# Autodesk Inventor assembly: front_panel
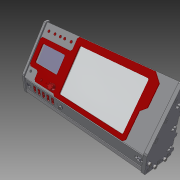
[picture p0: Inventor's stored thumbnail of the model, 180x180]
Saved by Autodesk Inventor 2014 (Build 180170000, 170)
## iProperties
Created: 2014-04-02
Part Number: front_panel
Document SubType Name: Assembly
Designer: buben
Author: buben
## Documents named in this file (20)
- C:\Users\buben\Documents\GitHub\bacon\inventor files\assemblies\front_panel.iam
- C:\Users\buben\Documents\GitHub\bacon\inventor files\printer parts\front_panel_brace_right.ipt
- C:\Users\buben\Documents\GitHub\bacon\inventor files\printer parts\front_panel_lcd.ipt
- C:\Users\buben\Documents\GitHub\bacon\inventor files\printer parts\front_panel_bottom.ipt
- C:\Users\buben\Documents\GitHub\bacon\inventor files\printer parts\front_panel_middle.ipt
- C:\Users\buben\Documents\GitHub\bacon\inventor files\printer parts\front_panel_brace_left.ipt
- C:\Users\buben\Documents\GitHub\bacon\inventor files\utils\washer_m4.ipt
- C:\Users\buben\Documents\Inventor\Content Center Files\R2014\en-US\ISO 4762(2)\ISO 4762 - M4 x 20ISO.ipt
- C:\Users\buben\Documents\Inventor\Content Center Files\R2014\en-US\ISO 7040\ISO 7040 - M4.ipt
- C:\Users\buben\Documents\GitHub\bacon\inventor files\printer parts\front_panel_brace_middle.ipt
- C:\Users\buben\Documents\GitHub\bacon\inventor files\utils\main_lcd_controller\lcd_controller.iam
- C:\Users\buben\Documents\GitHub\bacon\inventor files\utils\main_lcd_push_button.ipt
- C:\Users\buben\Documents\GitHub\bacon\inventor files\3rd party components\USB socket\Imported Components\USB-Socket\USB-Socket.ipt
- C:\Users\buben\Documents\GitHub\bacon\inventor files\utils\ramps_smart_controller\controler.iam
- C:\Users\buben\Documents\GitHub\bacon\inventor files\utils\controller_lcd_cover_glass.ipt
- C:\Users\buben\Documents\GitHub\bacon\inventor files\utils\main_lcd_panel.ipt
- C:\Users\buben\Documents\GitHub\bacon\inventor files\utils\main_lcd_cover_glass.ipt
- C:\Users\buben\Documents\GitHub\bacon\inventor files\utils\front_panel_frame.ipt
- C:\Users\buben\Documents\GitHub\bacon\inventor files\utils\controller_push_button.ipt
- C:\Users\buben\Documents\GitHub\bacon\inventor files\utils\rotary_encoder_cnob.ipt
## Components (56 placed, 19 different names)
1. front_panel_brace_right:1 — Flush:1, Mate:1, Mate:2, Mate:3, Mate:4, Mate:5, Mate:6, Mate:7, Mate:8, Mate:9, Flush:2, Flush:3, Mate:14, Mate:15, Mate:16, Mate:17, Mate:18, Mate:19
2. front_panel_lcd:1 — Mate:3, Mate:4, Mate:5, Mate:10, Mate:11, Mate:12, Mate:44, Angle:1, Mate:45, Mate:46, Mate:47, Mate:48, Mate:49, Mate:50, Flush:4, Mate:59, Mate:60, Flush:5, Mate:61, Mate:62, Mate:63, Flush:6, Mate:64, Flush:7, Mate:65, Mate:66, Mate:79, Mate:80
3. front_panel_bottom:1 — Mate:6, Mate:7, Mate:8, Mate:13, Mate:21, Mate:22, Mate:42, Mate:43, Mate:69, Mate:70
4. front_panel_middle:1 — Mate:9, Flush:2, Mate:10, Mate:20, Mate:41, Mate:56, Mate:57, Mate:58, Mate:67, Mate:68
5. front_panel_brace_left:1 — Mate:11, Mate:12, Mate:13
6. CSN 02 1702 B B 4,3:1 — Mate:15, Mate:18, Insert:2
7. CSN 02 1702 B B 4,3:2 — Mate:14, Mate:19, Insert:3
8. CSN 02 1702 B B 4,3:3 — Mate:16, Mate:17, Insert:1
9. CSN 02 1702 B B 4,3:4 — Mate:21, Mate:24, Mate:28
10. CSN 02 1702 B B 4,3:5 — Mate:22, Mate:25, Mate:30
11. CSN 02 1702 B B 4,3:6 — Mate:20, Mate:23, Mate:26
12. ISO 4762 M4 x 20:1 — Insert:1, Mate:23, Mate:27
13. ISO 4762 M4 x 20:2 — Insert:2, Mate:24, Mate:29
14. ISO 4762 M4 x 20:3 — Insert:3, Mate:25, Mate:31
15. DIN EN ISO 7040 M4:1 — Mate:30, Mate:31
16. DIN EN ISO 7040 M4:2 — Mate:28, Mate:29
17. DIN EN ISO 7040 M4:3 — Mate:26, Mate:27
18. CSN 02 1702 B B 4,3:7 — Insert:5
19. CSN 02 1702 B B 4,3:8 — Insert:6
20. CSN 02 1702 B B 4,3:9 — Insert:4
21. CSN 02 1702 B B 4,3:10 — Mate:33, Mate:38
22. CSN 02 1702 B B 4,3:11 — Mate:34, Mate:36
23. CSN 02 1702 B B 4,3:12 — Mate:32, Mate:40
24. ISO 4762 M4 x 20:4 — Mate:32, Insert:4, Mate:39
25. ISO 4762 M4 x 20:5 — Mate:33, Insert:5, Mate:37
26. ISO 4762 M4 x 20:6 — Mate:34, Insert:6, Mate:35
27. DIN EN ISO 7040 M4:4 — Mate:35, Mate:36
28. DIN EN ISO 7040 M4:5 — Mate:37, Mate:38
29. DIN EN ISO 7040 M4:6 — Mate:39, Mate:40
30. front_panel_brace_middle:1 — Mate:41, Mate:42, Mate:43, Mate:71, Mate:73
31. lcd_controller:1 [sub-assembly] — Mate:44, Angle:1, Mate:45, Mate:51, Mate:52, Mate:53, Mate:54, Mate:55
32. main_lcd_push_button:1 — Mate:46, Mate:55
33. main_lcd_push_button:2 — Mate:47, Mate:54
34. main_lcd_push_button:3 — Mate:48, Mate:53
35. main_lcd_push_button:4 — Mate:49, Mate:52
36. main_lcd_push_button:5 — Mate:50, Mate:51
37. controler:1 [sub-assembly] — Flush:4, Mate:59, Mate:60, Mate:81, Mate:82
38. controller_lcd_cover_glass:1 — Flush:5, Mate:61, Mate:62
39. main_lcd_panel:1 — Mate:63, Flush:6, Mate:64, Flush:8, Flush:9
40. main_lcd_cover_glass:1 — Flush:7, Mate:65, Mate:66
41. CSN 02 1702 B B 4,3:13 — Mate:71, Mate:72, Mate:75
42. CSN 02 1702 B B 4,3:14 — Mate:69, Mate:70, Insert:8
43. CSN 02 1702 B B 4,3:15 — Mate:67, Mate:68, Insert:7
44. CSN 02 1702 B B 4,3:16 — Mate:73, Mate:74, Mate:77
45. ISO 4762 M4 x 20:7 — Insert:8, Mate:72, Mate:76
46. ISO 4762 M4 x 20:8 — Insert:7, Mate:74, Mate:78
47. DIN EN ISO 7040 M4:7 — Mate:75, Mate:76
48. DIN EN ISO 7040 M4:8 — Mate:77, Mate:78
49. front_panel_frame:1 — Mate:79, Flush:8, Flush:9, Mate:83
50. controller_push_button:1 — Mate:80, Mate:81
51. rotary_encoder_cnob:1 — Mate:82, Mate:83
52. USB-Socket:1 — Mate:56, Mate:57, Mate:58
53. USB-Socket:2
54. USB-Socket:3
55. USB-Socket:4
56. USB-Socket:5
## Component patterns: (5 elements, first: USB-Socket:1)
## Relationships (101: Mate 83, Flush 9, Insert 8, Angle 1)
- Flush:1: front_panel_brace_right:1
- Mate:1: front_panel_brace_right:1
- Mate:2: front_panel_brace_right:1
- Mate:3: front_panel_brace_right:1 ↔ front_panel_lcd:1
- Mate:4: front_panel_brace_right:1 ↔ front_panel_lcd:1
- Mate:5: front_panel_brace_right:1 ↔ front_panel_lcd:1
- Mate:6: front_panel_brace_right:1 ↔ front_panel_bottom:1
- Mate:7: front_panel_brace_right:1 ↔ front_panel_bottom:1
- Mate:8: front_panel_brace_right:1 ↔ front_panel_bottom:1
- Mate:9: front_panel_brace_right:1 ↔ front_panel_middle:1
- Flush:2 (3 mm): front_panel_brace_right:1 ↔ front_panel_middle:1
- Mate:10 (1 mm): front_panel_lcd:1 ↔ front_panel_middle:1
- Mate:11: front_panel_lcd:1 ↔ front_panel_brace_left:1
- Mate:12: front_panel_lcd:1 ↔ front_panel_brace_left:1
- Mate:13: front_panel_bottom:1 ↔ front_panel_brace_left:1
- Flush:3 (150 mm): front_panel_brace_right:1
- Mate:14: front_panel_brace_right:1 ↔ CSN 02 1702 B B 4,3:2
- Mate:15: front_panel_brace_right:1 ↔ CSN 02 1702 B B 4,3:1
- Mate:16: front_panel_brace_right:1 ↔ CSN 02 1702 B B 4,3:3
- Mate:17: front_panel_brace_right:1 ↔ CSN 02 1702 B B 4,3:3
- Mate:18: front_panel_brace_right:1 ↔ CSN 02 1702 B B 4,3:1
- Mate:19: front_panel_brace_right:1 ↔ CSN 02 1702 B B 4,3:2
- Mate:20: front_panel_middle:1 ↔ CSN 02 1702 B B 4,3:6
- Mate:21: front_panel_bottom:1 ↔ CSN 02 1702 B B 4,3:4
- Mate:22: front_panel_bottom:1 ↔ CSN 02 1702 B B 4,3:5
- Insert:1: CSN 02 1702 B B 4,3:3 ↔ ISO 4762 M4 x 20:1
- Insert:2: CSN 02 1702 B B 4,3:1 ↔ ISO 4762 M4 x 20:2
- Insert:3: CSN 02 1702 B B 4,3:2 ↔ ISO 4762 M4 x 20:3
- Mate:23: CSN 02 1702 B B 4,3:6 ↔ ISO 4762 M4 x 20:1
- Mate:24: CSN 02 1702 B B 4,3:4 ↔ ISO 4762 M4 x 20:2
- Mate:25: CSN 02 1702 B B 4,3:5 ↔ ISO 4762 M4 x 20:3
- Mate:26: CSN 02 1702 B B 4,3:6 ↔ DIN EN ISO 7040 M4:3
- Mate:27: ISO 4762 M4 x 20:1 ↔ DIN EN ISO 7040 M4:3
- Mate:28: CSN 02 1702 B B 4,3:4 ↔ DIN EN ISO 7040 M4:2
- Mate:29: ISO 4762 M4 x 20:2 ↔ DIN EN ISO 7040 M4:2
- Mate:30: CSN 02 1702 B B 4,3:5 ↔ DIN EN ISO 7040 M4:1
- Mate:31: ISO 4762 M4 x 20:3 ↔ DIN EN ISO 7040 M4:1
- Mate:32: CSN 02 1702 B B 4,3:12 ↔ ISO 4762 M4 x 20:4
- Insert:4: CSN 02 1702 B B 4,3:9 ↔ ISO 4762 M4 x 20:4
- Mate:33: CSN 02 1702 B B 4,3:10 ↔ ISO 4762 M4 x 20:5
- Insert:5: CSN 02 1702 B B 4,3:7 ↔ ISO 4762 M4 x 20:5
- Mate:34: CSN 02 1702 B B 4,3:11 ↔ ISO 4762 M4 x 20:6
- Insert:6: CSN 02 1702 B B 4,3:8 ↔ ISO 4762 M4 x 20:6
- Mate:35: ISO 4762 M4 x 20:6 ↔ DIN EN ISO 7040 M4:4
- Mate:36: CSN 02 1702 B B 4,3:11 ↔ DIN EN ISO 7040 M4:4
- Mate:37: ISO 4762 M4 x 20:5 ↔ DIN EN ISO 7040 M4:5
- Mate:38: CSN 02 1702 B B 4,3:10 ↔ DIN EN ISO 7040 M4:5
- Mate:39: ISO 4762 M4 x 20:4 ↔ DIN EN ISO 7040 M4:6
- Mate:40: CSN 02 1702 B B 4,3:12 ↔ DIN EN ISO 7040 M4:6
- Mate:41: front_panel_middle:1 ↔ front_panel_brace_middle:1
- Mate:42: front_panel_bottom:1 ↔ front_panel_brace_middle:1
- Mate:43: front_panel_bottom:1 ↔ front_panel_brace_middle:1
- Mate:44: front_panel_lcd:1 ↔ lcd_controller:1
- Angle:1 (0 deg): front_panel_lcd:1 ↔ lcd_controller:1
- Mate:45 (6 mm): front_panel_lcd:1 ↔ lcd_controller:1
- Mate:46: front_panel_lcd:1 ↔ main_lcd_push_button:1
- Mate:47: front_panel_lcd:1 ↔ main_lcd_push_button:2
- Mate:48: front_panel_lcd:1 ↔ main_lcd_push_button:3
- Mate:49: front_panel_lcd:1 ↔ main_lcd_push_button:4
- Mate:50: front_panel_lcd:1 ↔ main_lcd_push_button:5
- Mate:51: lcd_controller:1 ↔ main_lcd_push_button:5
- Mate:52: lcd_controller:1 ↔ main_lcd_push_button:4
- Mate:53: lcd_controller:1 ↔ main_lcd_push_button:3
- Mate:54: lcd_controller:1 ↔ main_lcd_push_button:2
- Mate:55: lcd_controller:1 ↔ main_lcd_push_button:1
- Mate:56: front_panel_middle:1 ↔ USB-Socket:1
- Mate:57 (0.5 mm): front_panel_middle:1 ↔ USB-Socket:1
- Mate:58 (0.5 mm): front_panel_middle:1 ↔ USB-Socket:1
- Flush:4 (2 mm): front_panel_lcd:1 ↔ controler:1
- Mate:59 (-0.7 mm): front_panel_lcd:1 ↔ controler:1
- Mate:60 (0.65 mm): front_panel_lcd:1 ↔ controler:1
- Flush:5: front_panel_lcd:1 ↔ controller_lcd_cover_glass:1
- Mate:61: front_panel_lcd:1 ↔ controller_lcd_cover_glass:1
- Mate:62: front_panel_lcd:1 ↔ controller_lcd_cover_glass:1
- Mate:63 (0.5 mm): front_panel_lcd:1 ↔ main_lcd_panel:1
- Flush:6 (2 mm): front_panel_lcd:1 ↔ main_lcd_panel:1
- Mate:64 (0.5 mm): front_panel_lcd:1 ↔ main_lcd_panel:1
- Flush:7: front_panel_lcd:1 ↔ main_lcd_cover_glass:1
- Mate:65: front_panel_lcd:1 ↔ main_lcd_cover_glass:1
- Mate:66: front_panel_lcd:1 ↔ main_lcd_cover_glass:1
- Mate:67: front_panel_middle:1 ↔ CSN 02 1702 B B 4,3:15
- Mate:68: front_panel_middle:1 ↔ CSN 02 1702 B B 4,3:15
- Mate:69: front_panel_bottom:1 ↔ CSN 02 1702 B B 4,3:14
- Mate:70: front_panel_bottom:1 ↔ CSN 02 1702 B B 4,3:14
- Insert:7: CSN 02 1702 B B 4,3:15 ↔ ISO 4762 M4 x 20:8
- Insert:8: CSN 02 1702 B B 4,3:14 ↔ ISO 4762 M4 x 20:7
- Mate:71: front_panel_brace_middle:1 ↔ CSN 02 1702 B B 4,3:13
- Mate:72: CSN 02 1702 B B 4,3:13 ↔ ISO 4762 M4 x 20:7
- Mate:73: front_panel_brace_middle:1 ↔ CSN 02 1702 B B 4,3:16
- Mate:74: CSN 02 1702 B B 4,3:16 ↔ ISO 4762 M4 x 20:8
- Mate:75: CSN 02 1702 B B 4,3:13 ↔ DIN EN ISO 7040 M4:7
- Mate:76: ISO 4762 M4 x 20:7 ↔ DIN EN ISO 7040 M4:7
- Mate:77: CSN 02 1702 B B 4,3:16 ↔ DIN EN ISO 7040 M4:8
- Mate:78: ISO 4762 M4 x 20:8 ↔ DIN EN ISO 7040 M4:8
- Mate:79: front_panel_lcd:1 ↔ front_panel_frame:1
- Flush:8: main_lcd_panel:1 ↔ front_panel_frame:1
- Flush:9: main_lcd_panel:1 ↔ front_panel_frame:1
- Mate:80: front_panel_lcd:1 ↔ controller_push_button:1
- Mate:81: controler:1 ↔ controller_push_button:1
- Mate:82: controler:1 ↔ rotary_encoder_cnob:1
- Mate:83 (1 mm): front_panel_frame:1 ↔ rotary_encoder_cnob:1
